# Autodesk Inventor assembly: mallet_aseembly
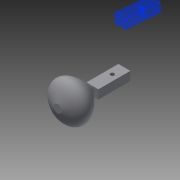
[picture p0: Inventor's stored thumbnail of the model, 180x180]
Saved by Autodesk Inventor 2015 (Build 190159000, 159)
## iProperties
Created: 2014-07-22
Part Number: mallet_aseembly
Document SubType Name: Assembly
Designer: shohei
Author: shohei
## Documents named in this file (3)
- C:\Users\shohei\Documents\Inventor\FufuPounder\mallet_aseembly.iam
- C:\Users\shohei\Documents\Inventor\FufuPounder\mallet_support.ipt
- C:\Users\shohei\Documents\Inventor\FufuPounder\mallet2.ipt
## Components (2 placed, 2 different names)
1. mallet_support:1 — Rotational:1
2. mallet2:1 — Rotational:1
## Relationships (1: RevoluteJoint 1)
- Rotational:1 [RevoluteJoint]: mallet_support:1 ↔ mallet2:1
